# Autodesk Inventor assembly: nhk_nc3
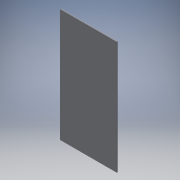
[picture p0: Inventor's stored thumbnail of the model, 180x180]
Saved by Autodesk Inventor 2019 (Build 230136000, 136)
## iProperties
Created: 2022-02-27
Part Number: nhk_nc3
Material: 一般
Document SubType Name: Assembly
Designer: yuta
Author: yuta
## Documents named in this file (3)
- C:\Users\yuta\Documents\NHK\nhk_nc3.iam
- C:\Users\yuta\Documents\NHK\NC.1.ipt
- C:\Users\yuta\Documents\NHK\nhk27.ipt
## Components (2 placed, 2 different names)
1. NC.1:1 — メイト:1, フラッシュ:1, フラッシュ:2
2. nhk27:1 — メイト:1, フラッシュ:1, フラッシュ:2
## Relationships (3: Flush 2, Mate 1)
- メイト:1 [Mate]: NC.1:1 ↔ nhk27:1
- フラッシュ:1 [Flush] (45 mm): NC.1:1 ↔ nhk27:1
- フラッシュ:2 [Flush] (30 mm): NC.1:1 ↔ nhk27:1
